# Autodesk Inventor assembly: quad1
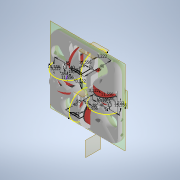
[picture p0: Inventor's stored thumbnail of the model, 180x180]
Saved by Autodesk Inventor 2020 (Build 240168000, 168)
## iProperties
Created: 2020-08-21
Part Number: quad1
Document SubType Name: Assembly
Designer: buran
Author: buran
## Documents named in this file (4)
- C:\Users\buran\Documents\erebos\motorCageAssembled.iam
- C:\Users\buran\Documents\erebos\motorCage.ipt
- C:\Users\buran\Documents\erebos\quadMotor.ipt
- C:\Users\buran\Documents\erebos\flyWheel.ipt
## Components (9 placed, 3 different names)
1. motorCage:1 — Rigid:1, Mate:1, Mate:2, Mate:3
2. quadMotor:1 — Mate:1
3. quadMotor:2 — Mate:2
4. quadMotor:3 — Rigid:1
5. quadMotor:4 — Mate:3
6. flyWheel:1
7. flyWheel:2
8. flyWheel:3
9. flyWheel:4
## Relationships (4: Mate 3, WeldJoint 1)
- Rigid:1 [WeldJoint]: motorCage:1 ↔ quadMotor:3
- Mate:1: motorCage:1 ↔ quadMotor:1
- Mate:2: motorCage:1 ↔ quadMotor:2
- Mate:3: motorCage:1 ↔ quadMotor:4
